# Autodesk Inventor assembly: New Assembly
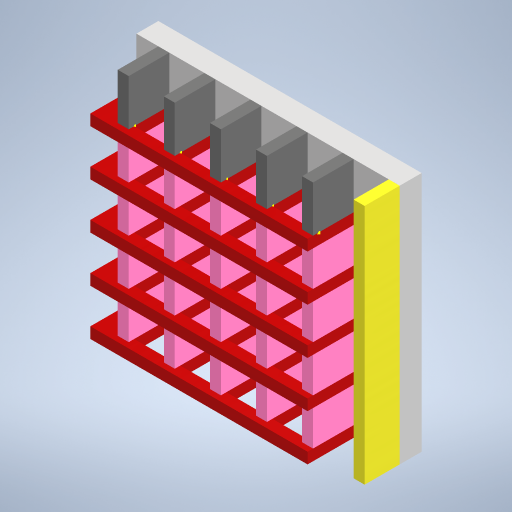
[picture p0: Inventor's stored thumbnail of the model, 512x512]
Saved by Autodesk Inventor 2024 (Build 280153000, 153)
## iProperties
Created: 2023-10-24
Part Number: New Assembly
Document SubType Name: Assembly
Designer: flynf
Author: flynf
## Documents named in this file (6)
- C:\Users\Owner\Desktop\SCHOOL\senior design\dotrix\CAD\New Assembly.iam
- C:\Users\Owner\Desktop\SCHOOL\senior design\dotrix\CAD\NewBackPlate.ipt
- C:\Users\Owner\Desktop\SCHOOL\senior design\dotrix\CAD\Side Plate.ipt
- C:\Users\Owner\Desktop\SCHOOL\senior design\dotrix\CAD\Spacer Sm.ipt
- C:\Users\Owner\Desktop\SCHOOL\senior design\dotrix\CAD\Spacer Bg.ipt
- C:\Users\Owner\Desktop\SCHOOL\senior design\dotrix\CAD\NewSlide.ipt
## Components (32 placed, 5 different names)
1. NewBackPlate:1 — Mate:3, Mate:4, Mate:5, Mate:6, Flush:3, Flush:4, Flush:5, Flush:6, Mate:7, Mate:8, Mate:9, Mate:10, Mate:11, Flush:7, Flush:8, Mate:12, Mate:13, Mate:14, Mate:15, Flush:9, Flush:10, Flush:11, Flush:12, Mate:16, Mate:17, Mate:18, Mate:19, Mate:20, Mate:21, Mate:22, Mate:23, Flush:13, Flush:14, Flush:15, Flush:16, Mate:24, Mate:25, Mate:26, Mate:27, Mate:28, Mate:29, Mate:30, Mate:31, Flush:17, Flush:18, Flush:19, Flush:20, Mate:32, Mate:33, Mate:34, Mate:35, Mate:36, Mate:37, Mate:38, Mate:39, Flush:21, Flush:22, Flush:23, Flush:24, Flush:25, Flush:26, Flush:27, Flush:28, Mate:40, Mate:41, Mate:42, Mate:43, Mate:44, Flush:29, Flush:30, Flush:31, Flush:32, Flush:33, Mate:45, Mate:46, Mate:47, Flush:34, Mate:48, Mate:49, Mate:50, Flush:35, Mate:51, Mate:52, Flush:36, Mate:53, Mate:54, Flush:37, Mate:55, Mate:56, Flush:38, Mate:57, Mate:58, Flush:39
2. Spacer Sm:1 — Mate:5, Flush:6, Mate:10
3. Spacer Sm:2 — Mate:4, Flush:4, Mate:8
4. Spacer Sm:3 — Mate:3, Flush:3, Mate:7
5. Spacer Sm:4 — Mate:6, Flush:5, Mate:9
6. Side Plate:1 — Mate:11, Flush:7, Flush:8
7. Spacer Sm:5 — Mate:15, Flush:9, Mate:16
8. Spacer Sm:6 — Mate:14, Flush:10, Mate:17
9. Spacer Sm:7 — Mate:13, Flush:11, Mate:18
10. Spacer Sm:8 — Mate:12, Flush:12, Mate:19
11. Spacer Sm:9 — Mate:23, Flush:13, Mate:24
12. Spacer Sm:10 — Mate:22, Flush:14, Mate:25
13. Spacer Sm:11 — Mate:21, Flush:15, Mate:26
14. Spacer Sm:12 — Mate:20, Flush:16, Mate:27
15. Spacer Sm:13 — Mate:31, Flush:20, Mate:32
16. Spacer Sm:14 — Mate:29, Flush:18, Mate:34
17. Spacer Sm:15 — Mate:30, Flush:19, Mate:33
18. Spacer Sm:16 — Mate:37, Flush:23, Flush:27
19. Spacer Sm:17 — Mate:39, Flush:21, Flush:25
20. Spacer Sm:18 — Mate:38, Flush:22, Flush:26
21. Spacer Sm:19 — Mate:28, Flush:17, Mate:35
22. Spacer Sm:20 — Mate:36, Flush:24, Flush:28
23. Spacer Bg:1 — Mate:40, Flush:29, Mate:45
24. Spacer Bg:2 — Mate:42, Flush:31, Mate:47
25. Spacer Bg:3 — Mate:43, Flush:32, Mate:48
26. Spacer Bg:4 — Mate:44, Flush:33, Flush:34
27. Spacer Bg:5 — Mate:41, Flush:30, Mate:46
28. NewSlide:1 — Mate:55, Mate:56, Flush:38
29. NewSlide:2 — Mate:53, Mate:54, Flush:37
30. NewSlide:3 — Mate:51, Mate:52, Flush:36
31. NewSlide:4 — Mate:49, Mate:50, Flush:35
32. NewSlide:5 — Mate:57, Mate:58, Flush:39
## Relationships (93: Mate 56, Flush 37)
- Mate:3: NewBackPlate:1 ↔ Spacer Sm:3
- Mate:4: NewBackPlate:1 ↔ Spacer Sm:2
- Mate:5: NewBackPlate:1 ↔ Spacer Sm:1
- Mate:6: NewBackPlate:1 ↔ Spacer Sm:4
- Flush:3: NewBackPlate:1 ↔ Spacer Sm:3
- Flush:4: NewBackPlate:1 ↔ Spacer Sm:2
- Flush:5: NewBackPlate:1 ↔ Spacer Sm:4
- Flush:6: NewBackPlate:1 ↔ Spacer Sm:1
- Mate:7 (40.64 mm): NewBackPlate:1 ↔ Spacer Sm:3
- Mate:8 (40.64 mm): NewBackPlate:1 ↔ Spacer Sm:2
- Mate:9 (40.64 mm): NewBackPlate:1 ↔ Spacer Sm:4
- Mate:10 (40.64 mm): NewBackPlate:1 ↔ Spacer Sm:1
- Mate:11: NewBackPlate:1 ↔ Side Plate:1
- Flush:7: NewBackPlate:1 ↔ Side Plate:1
- Flush:8: NewBackPlate:1 ↔ Side Plate:1
- Mate:12: NewBackPlate:1 ↔ Spacer Sm:8
- Mate:13: NewBackPlate:1 ↔ Spacer Sm:7
- Mate:14: NewBackPlate:1 ↔ Spacer Sm:6
- Mate:15: NewBackPlate:1 ↔ Spacer Sm:5
- Flush:9: NewBackPlate:1 ↔ Spacer Sm:5
- Flush:10: NewBackPlate:1 ↔ Spacer Sm:6
- Flush:11: NewBackPlate:1 ↔ Spacer Sm:7
- Flush:12: NewBackPlate:1 ↔ Spacer Sm:8
- Mate:16 (93.98 mm): NewBackPlate:1 ↔ Spacer Sm:5
- Mate:17 (93.98 mm): NewBackPlate:1 ↔ Spacer Sm:6
- Mate:18 (93.98 mm): NewBackPlate:1 ↔ Spacer Sm:7
- Mate:19 (93.98 mm): NewBackPlate:1 ↔ Spacer Sm:8
- Mate:20: NewBackPlate:1 ↔ Spacer Sm:12
- Mate:21: NewBackPlate:1 ↔ Spacer Sm:11
- Mate:22: NewBackPlate:1 ↔ Spacer Sm:10
- Mate:23: NewBackPlate:1 ↔ Spacer Sm:9
- Flush:13: NewBackPlate:1 ↔ Spacer Sm:9
- Flush:14: NewBackPlate:1 ↔ Spacer Sm:10
- Flush:15: NewBackPlate:1 ↔ Spacer Sm:11
- Flush:16: NewBackPlate:1 ↔ Spacer Sm:12
- Mate:24 (147.32 mm): NewBackPlate:1 ↔ Spacer Sm:9
- Mate:25 (147.32 mm): NewBackPlate:1 ↔ Spacer Sm:10
- Mate:26 (147.32 mm): NewBackPlate:1 ↔ Spacer Sm:11
- Mate:27 (147.32 mm): NewBackPlate:1 ↔ Spacer Sm:12
- Mate:28: NewBackPlate:1 ↔ Spacer Sm:19
- Mate:29: NewBackPlate:1 ↔ Spacer Sm:14
- Mate:30: NewBackPlate:1 ↔ Spacer Sm:15
- Mate:31: NewBackPlate:1 ↔ Spacer Sm:13
- Flush:17: NewBackPlate:1 ↔ Spacer Sm:19
- Flush:18: NewBackPlate:1 ↔ Spacer Sm:14
- Flush:19: NewBackPlate:1 ↔ Spacer Sm:15
- Flush:20: NewBackPlate:1 ↔ Spacer Sm:13
- Mate:32 (200.66 mm): NewBackPlate:1 ↔ Spacer Sm:13
- Mate:33 (200.66 mm): NewBackPlate:1 ↔ Spacer Sm:15
- Mate:34 (200.66 mm): NewBackPlate:1 ↔ Spacer Sm:14
- Mate:35 (200.66 mm): NewBackPlate:1 ↔ Spacer Sm:19
- Mate:36: NewBackPlate:1 ↔ Spacer Sm:20
- Mate:37: NewBackPlate:1 ↔ Spacer Sm:16
- Mate:38: NewBackPlate:1 ↔ Spacer Sm:18
- Mate:39: NewBackPlate:1 ↔ Spacer Sm:17
- Flush:21: NewBackPlate:1 ↔ Spacer Sm:17
- Flush:22: NewBackPlate:1 ↔ Spacer Sm:18
- Flush:23: NewBackPlate:1 ↔ Spacer Sm:16
- Flush:24: NewBackPlate:1 ↔ Spacer Sm:20
- Flush:25: NewBackPlate:1 ↔ Spacer Sm:17
- Flush:26: NewBackPlate:1 ↔ Spacer Sm:18
- Flush:27: NewBackPlate:1 ↔ Spacer Sm:16
- Flush:28: NewBackPlate:1 ↔ Spacer Sm:20
- Mate:40: NewBackPlate:1 ↔ Spacer Bg:1
- Mate:41: NewBackPlate:1 ↔ Spacer Bg:5
- Mate:42: NewBackPlate:1 ↔ Spacer Bg:2
- Mate:43: NewBackPlate:1 ↔ Spacer Bg:3
- Mate:44: NewBackPlate:1 ↔ Spacer Bg:4
- Flush:29: NewBackPlate:1 ↔ Spacer Bg:1
- Flush:30: NewBackPlate:1 ↔ Spacer Bg:5
- Flush:31: NewBackPlate:1 ↔ Spacer Bg:2
- Flush:32: NewBackPlate:1 ↔ Spacer Bg:3
- Flush:33: NewBackPlate:1 ↔ Spacer Bg:4
- Mate:45 (40.64 mm): NewBackPlate:1 ↔ Spacer Bg:1
- Mate:46 (93.98 mm): NewBackPlate:1 ↔ Spacer Bg:5
- Mate:47 (147.32 mm): NewBackPlate:1 ↔ Spacer Bg:2
- Flush:34: NewBackPlate:1 ↔ Spacer Bg:4
- Mate:48 (200.66 mm): NewBackPlate:1 ↔ Spacer Bg:3
- Mate:49: NewBackPlate:1 ↔ NewSlide:4
- Mate:50: NewBackPlate:1 ↔ NewSlide:4
- Flush:35 (-25.4 mm): NewBackPlate:1 ↔ NewSlide:4
- Mate:51: NewBackPlate:1 ↔ NewSlide:3
- Mate:52: NewBackPlate:1 ↔ NewSlide:3
- Flush:36 (-25.4 mm): NewBackPlate:1 ↔ NewSlide:3
- Mate:53: NewBackPlate:1 ↔ NewSlide:2
- Mate:54: NewBackPlate:1 ↔ NewSlide:2
- Flush:37 (-25.4 mm): NewBackPlate:1 ↔ NewSlide:2
- Mate:55: NewBackPlate:1 ↔ NewSlide:1
- Mate:56: NewBackPlate:1 ↔ NewSlide:1
- Flush:38 (-25.4 mm): NewBackPlate:1 ↔ NewSlide:1
- Mate:57: NewBackPlate:1 ↔ NewSlide:5
- Mate:58: NewBackPlate:1 ↔ NewSlide:5
- Flush:39 (-25.4 mm): NewBackPlate:1 ↔ NewSlide:5
